# Autodesk Inventor assembly: Portalfraese_V2_Z-Axis
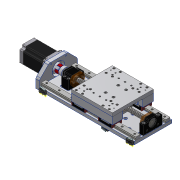
[picture p0: Inventor's stored thumbnail of the model, 180x180]
Saved by Autodesk Inventor 2016 (Build 200138000, 138)
## iProperties
Created: 2015-07-20
Part Number: Portalfraese_V2_Z-Axis
Document SubType Name: Assembly
Mass: 4544.64 g
Surface Area: 3288.98 cm^2
Volume: 1436.27 cm^3
Density: 3.16419 g/cm^3
## Documents named in this file (22)
- E:\GitHub\CNC-Router_Z-Axis\CNC-Router_Z-Axis.iam
- E:\GitHub\CNC-Router_Z-Axis\Linearfuehrung Bosch Rexroth R0442.iam
- E:\GitHub\CNC-Router_Z-Axis\ISSOKU_Ballscrew_D12x160_05_590104-13.iam
- E:\GitHub\CNC-Router_Z-Axis\Grundplatte.ipt
- E:\GitHub\Buy-Parts\Stepper_Nema23_23HS33-4008S.ipt
- E:\GitHub\CNC-Router_Z-Axis\Motorhalterung.ipt
- E:\GitHub\Buy-Parts\Klauenkupplung_d6-35_d8.ipt
- E:\GitHub\CNC-Router_Z-Axis\Schlitten.iam
- E:\GitHub\Standard-Parts\Zyl-Schr_ISO 4762 - M4 x 12_St-Vzkt.ipt
- E:\GitHub\Standard-Parts\Zyl-Schr_ISO 4762 - M3 x 35_INOX.ipt
- E:\GitHub\Standard-Parts\Zyl-Schr_ISO 4762 - M3 x 10_St-Vzkt.ipt
- E:\GitHub\Standard-Parts\U-Scheibe_ISO 7089 - 4 - 140 HV_St-Vzkt.ipt
- E:\GitHub\Standard-Parts\U-Scheibe_ISO 7089 - 6 - 140 HV_St-Vzkt.ipt
- E:\GitHub\Standard-Parts\Zyl-Schr_ISO 4762 - M6 x 20_St-Vzkt.ipt
- E:\GitHub\Standard-Parts\Zyl-Schr_ISO 4762 - M4 x 30_St-Vzkt.ipt
- E:\GitHub\Standard-Parts\Zyl-Schr_ISO 4762 - M5 x 30_St-Vzkt.ipt
- E:\GitHub\Buy-Parts\Microswitch Dongnan KW4A (S).ipt
- E:\GitHub\Buy-Parts\Klebesockel_HC-101SBK.ipt
- E:\GitHub\Buy-Parts\Micro_Mate-N-Lok_TE-Connectivity_3mm_1x4_Female.iam
- E:\GitHub\Buy-Parts\Micro_Mate-N-Lok_TE-Connectivity_3mm_2x2_Female.iam
- E:\GitHub\CNC-Router_Z-Axis\Zyl-Schr_ISO 4762 - M2 x 10_St-B.iam
- E:\GitHub\Standard-Parts\U-Scheibe_DIN 125 - A 2.2.ipt
## Components (86 placed, 21 different names)
1. ISSOKU_Ballscrew_D12x160_05_590104-13:1 [sub-assembly] — Mate:3, Mate:5, Mate:8, Insert:1, Mate:16, Mate:17, Flush:12, Mate:22, Insert:52, Insert:53, Insert:54, Insert:55, Insert:56, Insert:57
2. Linearfuehrung Bosch Rexroth R0442:1 [sub-assembly] — Mate:4, Flush:8, Mate:21, Mate:23, Mate:27, Insert:24, Insert:25, Insert:26, Insert:27, Insert:36, Insert:37, Insert:38, Insert:39
3. Linearfuehrung Bosch Rexroth R0442:2 [sub-assembly] — Mate:24, Mate:26, Mate:28, Mate:29, Mate:30, Insert:28, Insert:29, Insert:30, Insert:31, Insert:32, Insert:33, Insert:34, Insert:35
4. Grundplatte:1 — Mate:3, Mate:4, Flush:8, Mate:5, Angle:1, Mate:10, Flush:10, Mate:16, Mate:23, Mate:24, Mate:28, Insert:58, Insert:59, Mate:31, Mate:32, Mate:33, Insert:60, Mate:34, Mate:35, Insert:61, Mate:36, Flush:13, Mate:37, Mate:38, Mate:39, Mate:40
5. Stepper_Nema23_23HS33-4008S:1 — Mate:8, Angle:1, Mate:11, Mate:14, Insert:40, Insert:41, Insert:42, Insert:43
6. Motorhalterung:1 — Mate:10, Mate:11, Flush:10, Mate:14, Mate:26, Insert:50, Insert:51, Flush:16, Flush:17
7. Klauenkupplung_d6-35_d8:1 — Insert:1
8. Schlitten:1 [sub-assembly] — Mate:17, Flush:12, Mate:21, Mate:22, Mate:27, Mate:29, Mate:30, Insert:8, Insert:9, Insert:10, Insert:11, Insert:12, Insert:13, Insert:14, Insert:15, Insert:16, Insert:17, Insert:18, Insert:19, Insert:20, Insert:21, Insert:22, Insert:23
9. Zyl-Schr_ISO 4762 - M4 x 12_St-Vzkt:1
10. Zyl-Schr_ISO 4762 - M4 x 12_St-Vzkt:2
11. Zyl-Schr_ISO 4762 - M4 x 12_St-Vzkt:3
12. Zyl-Schr_ISO 4762 - M4 x 12_St-Vzkt:4
13. Zyl-Schr_ISO 4762 - M3 x 35_INOX:1 — Insert:8
14. Zyl-Schr_ISO 4762 - M3 x 35_INOX:2 — Insert:9
15. Zyl-Schr_ISO 4762 - M3 x 35_INOX:3 — Insert:11
16. Zyl-Schr_ISO 4762 - M3 x 35_INOX:4 — Insert:13
17. Zyl-Schr_ISO 4762 - M3 x 35_INOX:5 — Insert:12
18. Zyl-Schr_ISO 4762 - M3 x 35_INOX:6 — Insert:10
19. Zyl-Schr_ISO 4762 - M3 x 35_INOX:7 — Insert:15
20. Zyl-Schr_ISO 4762 - M3 x 35_INOX:8 — Insert:16
21. Zyl-Schr_ISO 4762 - M3 x 35_INOX:9 — Insert:14
22. Zyl-Schr_ISO 4762 - M3 x 35_INOX:10 — Insert:19
23. Zyl-Schr_ISO 4762 - M3 x 35_INOX:11 — Insert:23
24. Zyl-Schr_ISO 4762 - M3 x 35_INOX:12 — Insert:17
25. Zyl-Schr_ISO 4762 - M3 x 35_INOX:13 — Insert:21
26. Zyl-Schr_ISO 4762 - M3 x 35_INOX:14 — Insert:22
27. Zyl-Schr_ISO 4762 - M3 x 35_INOX:15 — Insert:18
28. Zyl-Schr_ISO 4762 - M3 x 35_INOX:16 — Insert:20
29. Zyl-Schr_ISO 4762 - M3 x 10_St-Vzkt:1 — Insert:28
30. Zyl-Schr_ISO 4762 - M3 x 10_St-Vzkt:2 — Insert:29
31. Zyl-Schr_ISO 4762 - M3 x 10_St-Vzkt:3 — Insert:30
32. Zyl-Schr_ISO 4762 - M3 x 10_St-Vzkt:4 — Insert:31
33. Zyl-Schr_ISO 4762 - M3 x 10_St-Vzkt:5 — Insert:32
34. Zyl-Schr_ISO 4762 - M3 x 10_St-Vzkt:6 — Insert:33
35. Zyl-Schr_ISO 4762 - M3 x 10_St-Vzkt:7 — Insert:34
36. Zyl-Schr_ISO 4762 - M3 x 10_St-Vzkt:8 — Insert:35
37. Zyl-Schr_ISO 4762 - M3 x 10_St-Vzkt:9 — Insert:24
38. Zyl-Schr_ISO 4762 - M3 x 10_St-Vzkt:10 — Insert:25
39. Zyl-Schr_ISO 4762 - M3 x 10_St-Vzkt:11 — Insert:26
40. Zyl-Schr_ISO 4762 - M3 x 10_St-Vzkt:12 — Insert:27
41. Zyl-Schr_ISO 4762 - M3 x 10_St-Vzkt:13 — Insert:36
42. Zyl-Schr_ISO 4762 - M3 x 10_St-Vzkt:14 — Insert:37
43. Zyl-Schr_ISO 4762 - M3 x 10_St-Vzkt:15 — Insert:38
44. Zyl-Schr_ISO 4762 - M3 x 10_St-Vzkt:16 — Insert:39
45. Zyl-Schr_ISO 4762 - M4 x 12_St-Vzkt:5 — Insert:44
46. U-Scheibe_ISO 7089 - 4 - 140 HV_St-Vzkt:1 — Insert:40, Insert:44
47. U-Scheibe_ISO 7089 - 4 - 140 HV_St-Vzkt:2 — Insert:41, Insert:45
48. U-Scheibe_ISO 7089 - 4 - 140 HV_St-Vzkt:3 — Insert:42, Insert:46
49. U-Scheibe_ISO 7089 - 4 - 140 HV_St-Vzkt:4 — Insert:43, Insert:47
50. Zyl-Schr_ISO 4762 - M4 x 12_St-Vzkt:6 — Insert:45
51. Zyl-Schr_ISO 4762 - M4 x 12_St-Vzkt:7 — Insert:46
52. Zyl-Schr_ISO 4762 - M4 x 12_St-Vzkt:8 — Insert:47
53. U-Scheibe_ISO 7089 - 6 - 140 HV_St-Vzkt:1 — Insert:48, Insert:50
54. Zyl-Schr_ISO 4762 - M6 x 20_St-Vzkt:1 — Insert:48
55. U-Scheibe_ISO 7089 - 6 - 140 HV_St-Vzkt:2 — Insert:51
56. Zyl-Schr_ISO 4762 - M6 x 20_St-Vzkt:2
57. Zyl-Schr_ISO 4762 - M4 x 30_St-Vzkt:1 — Insert:52
58. Zyl-Schr_ISO 4762 - M4 x 30_St-Vzkt:2 — Insert:53
59. Zyl-Schr_ISO 4762 - M4 x 30_St-Vzkt:3 — Insert:54
60. Zyl-Schr_ISO 4762 - M4 x 30_St-Vzkt:4 — Insert:55
61. Zyl-Schr_ISO 4762 - M5 x 30_St-Vzkt:1 — Insert:56
62. Zyl-Schr_ISO 4762 - M5 x 30_St-Vzkt:2 — Insert:57
63. Microswitch Dongnan KW4A (S):1 — Mate:35, Insert:61, Insert:68, Insert:69
64. Microswitch Dongnan KW4A (S):2 — Insert:60, Mate:34, Insert:66, Insert:67
65. Microswitch Dongnan KW4A (S):3 — Insert:58, Mate:32, Mate:33, Insert:74, Insert:75
66. Microswitch Dongnan KW4A (S):4 — Insert:59, Mate:31, Insert:76, Insert:77
67. Klebesockel_HC-101SBK:1 — Mate:36, Flush:13, Mate:37
68. Micro_Mate-N-Lok_TE-Connectivity_3mm_1x4_Female:1 [sub-assembly] — Mate:39, Mate:41, Mate:42, Flush:14, Flush:15
69. Micro_Mate-N-Lok_TE-Connectivity_3mm_2x2_Female:1 [sub-assembly] — Mate:40, Mate:42, Flush:14, Flush:16, Flush:17
70. Micro_Mate-N-Lok_TE-Connectivity_3mm_1x4_Female:2 [sub-assembly] — Mate:38, Mate:41, Flush:15
71. Zyl-Schr_ISO 4762 - M2 x 10_St-B:1 [sub-assembly] — Insert:62
72. U-Scheibe_DIN 125 - A 2.2:1 — Insert:62, Insert:67
73. Zyl-Schr_ISO 4762 - M2 x 10_St-B:2 [sub-assembly]
74. U-Scheibe_DIN 125 - A 2.2:2 — Insert:66
75. Zyl-Schr_ISO 4762 - M2 x 10_St-B:3 [sub-assembly]
76. U-Scheibe_DIN 125 - A 2.2:3 — Insert:68
77. Zyl-Schr_ISO 4762 - M2 x 10_St-B:4 [sub-assembly]
78. U-Scheibe_DIN 125 - A 2.2:4 — Insert:69
79. Zyl-Schr_ISO 4762 - M2 x 10_St-B:5 [sub-assembly]
80. U-Scheibe_DIN 125 - A 2.2:5 — Insert:74
81. Zyl-Schr_ISO 4762 - M2 x 10_St-B:6 [sub-assembly]
82. U-Scheibe_DIN 125 - A 2.2:6 — Insert:75
83. Zyl-Schr_ISO 4762 - M2 x 10_St-B:7 [sub-assembly]
84. U-Scheibe_DIN 125 - A 2.2:7 — Insert:76
85. Zyl-Schr_ISO 4762 - M2 x 10_St-B:8 [sub-assembly]
86. U-Scheibe_DIN 125 - A 2.2:8 — Insert:77
## Relationships (114: Insert 75, Mate 30, Flush 8, Angle 1)
- Mate:3: ISSOKU_Ballscrew_D12x160_05_590104-13:1 ↔ Grundplatte:1
- Mate:4: Linearfuehrung Bosch Rexroth R0442:1 ↔ Grundplatte:1
- Flush:8: Linearfuehrung Bosch Rexroth R0442:1 ↔ Grundplatte:1
- Mate:5 (3 mm): ISSOKU_Ballscrew_D12x160_05_590104-13:1 ↔ Grundplatte:1
- Mate:8: ISSOKU_Ballscrew_D12x160_05_590104-13:1 ↔ Stepper_Nema23_23HS33-4008S:1
- Angle:1 (0 deg): Grundplatte:1 ↔ Stepper_Nema23_23HS33-4008S:1
- Mate:10: Grundplatte:1 ↔ Motorhalterung:1
- Mate:11: Stepper_Nema23_23HS33-4008S:1 ↔ Motorhalterung:1
- Flush:10: Grundplatte:1 ↔ Motorhalterung:1
- Insert:1 (1.5 mm): ISSOKU_Ballscrew_D12x160_05_590104-13:1 ↔ Klauenkupplung_d6-35_d8:1
- Mate:14: Stepper_Nema23_23HS33-4008S:1 ↔ Motorhalterung:1
- Mate:16: ISSOKU_Ballscrew_D12x160_05_590104-13:1 ↔ Grundplatte:1
- Mate:17: ISSOKU_Ballscrew_D12x160_05_590104-13:1 ↔ Schlitten:1
- Flush:12: ISSOKU_Ballscrew_D12x160_05_590104-13:1 ↔ Schlitten:1
- Mate:21: Linearfuehrung Bosch Rexroth R0442:1 ↔ Schlitten:1
- Mate:22: ISSOKU_Ballscrew_D12x160_05_590104-13:1 ↔ Schlitten:1
- Mate:23: Linearfuehrung Bosch Rexroth R0442:1 ↔ Grundplatte:1
- Mate:24: Linearfuehrung Bosch Rexroth R0442:2 ↔ Grundplatte:1
- Mate:26: Linearfuehrung Bosch Rexroth R0442:2 ↔ Motorhalterung:1
- Mate:27: Linearfuehrung Bosch Rexroth R0442:1 ↔ Schlitten:1
- Mate:28: Linearfuehrung Bosch Rexroth R0442:2 ↔ Grundplatte:1
- Mate:29: Linearfuehrung Bosch Rexroth R0442:2 ↔ Schlitten:1
- Mate:30: Linearfuehrung Bosch Rexroth R0442:2 ↔ Schlitten:1
- [Insert]: Schlitten:1 ↔ Zyl-Schr_ISO 4762 - M4 x 12_St-Vzkt:1
- [Insert]: Schlitten:1 ↔ Zyl-Schr_ISO 4762 - M4 x 12_St-Vzkt:2
- [Insert]: Schlitten:1 ↔ Zyl-Schr_ISO 4762 - M4 x 12_St-Vzkt:4
- [Insert]: Schlitten:1 ↔ Zyl-Schr_ISO 4762 - M4 x 12_St-Vzkt:3
- Insert:8: Schlitten:1 ↔ Zyl-Schr_ISO 4762 - M3 x 35_INOX:1
- Insert:9: Schlitten:1 ↔ Zyl-Schr_ISO 4762 - M3 x 35_INOX:2
- Insert:10: Schlitten:1 ↔ Zyl-Schr_ISO 4762 - M3 x 35_INOX:6
- Insert:11: Schlitten:1 ↔ Zyl-Schr_ISO 4762 - M3 x 35_INOX:3
- Insert:12: Schlitten:1 ↔ Zyl-Schr_ISO 4762 - M3 x 35_INOX:5
- Insert:13: Schlitten:1 ↔ Zyl-Schr_ISO 4762 - M3 x 35_INOX:4
- Insert:14: Schlitten:1 ↔ Zyl-Schr_ISO 4762 - M3 x 35_INOX:9
- Insert:15: Schlitten:1 ↔ Zyl-Schr_ISO 4762 - M3 x 35_INOX:7
- Insert:16: Schlitten:1 ↔ Zyl-Schr_ISO 4762 - M3 x 35_INOX:8
- Insert:17: Schlitten:1 ↔ Zyl-Schr_ISO 4762 - M3 x 35_INOX:12
- Insert:18: Schlitten:1 ↔ Zyl-Schr_ISO 4762 - M3 x 35_INOX:15
- Insert:19: Schlitten:1 ↔ Zyl-Schr_ISO 4762 - M3 x 35_INOX:10
- Insert:20: Schlitten:1 ↔ Zyl-Schr_ISO 4762 - M3 x 35_INOX:16
- Insert:21: Schlitten:1 ↔ Zyl-Schr_ISO 4762 - M3 x 35_INOX:13
- Insert:22: Schlitten:1 ↔ Zyl-Schr_ISO 4762 - M3 x 35_INOX:14
- Insert:23: Schlitten:1 ↔ Zyl-Schr_ISO 4762 - M3 x 35_INOX:11
- Insert:24: Linearfuehrung Bosch Rexroth R0442:1 ↔ Zyl-Schr_ISO 4762 - M3 x 10_St-Vzkt:9
- Insert:25: Linearfuehrung Bosch Rexroth R0442:1 ↔ Zyl-Schr_ISO 4762 - M3 x 10_St-Vzkt:10
- Insert:26: Linearfuehrung Bosch Rexroth R0442:1 ↔ Zyl-Schr_ISO 4762 - M3 x 10_St-Vzkt:11
- Insert:27: Linearfuehrung Bosch Rexroth R0442:1 ↔ Zyl-Schr_ISO 4762 - M3 x 10_St-Vzkt:12
- Insert:28: Linearfuehrung Bosch Rexroth R0442:2 ↔ Zyl-Schr_ISO 4762 - M3 x 10_St-Vzkt:1
- Insert:29: Linearfuehrung Bosch Rexroth R0442:2 ↔ Zyl-Schr_ISO 4762 - M3 x 10_St-Vzkt:2
- Insert:30: Linearfuehrung Bosch Rexroth R0442:2 ↔ Zyl-Schr_ISO 4762 - M3 x 10_St-Vzkt:3
- Insert:31: Linearfuehrung Bosch Rexroth R0442:2 ↔ Zyl-Schr_ISO 4762 - M3 x 10_St-Vzkt:4
- Insert:32: Linearfuehrung Bosch Rexroth R0442:2 ↔ Zyl-Schr_ISO 4762 - M3 x 10_St-Vzkt:5
- Insert:33: Linearfuehrung Bosch Rexroth R0442:2 ↔ Zyl-Schr_ISO 4762 - M3 x 10_St-Vzkt:6
- Insert:34: Linearfuehrung Bosch Rexroth R0442:2 ↔ Zyl-Schr_ISO 4762 - M3 x 10_St-Vzkt:7
- Insert:35: Linearfuehrung Bosch Rexroth R0442:2 ↔ Zyl-Schr_ISO 4762 - M3 x 10_St-Vzkt:8
- Insert:36: Linearfuehrung Bosch Rexroth R0442:1 ↔ Zyl-Schr_ISO 4762 - M3 x 10_St-Vzkt:13
- Insert:37: Linearfuehrung Bosch Rexroth R0442:1 ↔ Zyl-Schr_ISO 4762 - M3 x 10_St-Vzkt:14
- Insert:38: Linearfuehrung Bosch Rexroth R0442:1 ↔ Zyl-Schr_ISO 4762 - M3 x 10_St-Vzkt:15
- Insert:39: Linearfuehrung Bosch Rexroth R0442:1 ↔ Zyl-Schr_ISO 4762 - M3 x 10_St-Vzkt:16
- Insert:40: Stepper_Nema23_23HS33-4008S:1 ↔ U-Scheibe_ISO 7089 - 4 - 140 HV_St-Vzkt:1
- Insert:41: Stepper_Nema23_23HS33-4008S:1 ↔ U-Scheibe_ISO 7089 - 4 - 140 HV_St-Vzkt:2
- Insert:42: Stepper_Nema23_23HS33-4008S:1 ↔ U-Scheibe_ISO 7089 - 4 - 140 HV_St-Vzkt:3
- Insert:43: Stepper_Nema23_23HS33-4008S:1 ↔ U-Scheibe_ISO 7089 - 4 - 140 HV_St-Vzkt:4
- Insert:44: Zyl-Schr_ISO 4762 - M4 x 12_St-Vzkt:5 ↔ U-Scheibe_ISO 7089 - 4 - 140 HV_St-Vzkt:1
- Insert:45: U-Scheibe_ISO 7089 - 4 - 140 HV_St-Vzkt:2 ↔ Zyl-Schr_ISO 4762 - M4 x 12_St-Vzkt:6
- Insert:46: U-Scheibe_ISO 7089 - 4 - 140 HV_St-Vzkt:3 ↔ Zyl-Schr_ISO 4762 - M4 x 12_St-Vzkt:7
- Insert:47: U-Scheibe_ISO 7089 - 4 - 140 HV_St-Vzkt:4 ↔ Zyl-Schr_ISO 4762 - M4 x 12_St-Vzkt:8
- Insert:48: U-Scheibe_ISO 7089 - 6 - 140 HV_St-Vzkt:1 ↔ Zyl-Schr_ISO 4762 - M6 x 20_St-Vzkt:1
- [Insert]: U-Scheibe_ISO 7089 - 6 - 140 HV_St-Vzkt:2 ↔ Zyl-Schr_ISO 4762 - M6 x 20_St-Vzkt:2
- Insert:50: Motorhalterung:1 ↔ U-Scheibe_ISO 7089 - 6 - 140 HV_St-Vzkt:1
- Insert:51: Motorhalterung:1 ↔ U-Scheibe_ISO 7089 - 6 - 140 HV_St-Vzkt:2
- Insert:52: ISSOKU_Ballscrew_D12x160_05_590104-13:1 ↔ Zyl-Schr_ISO 4762 - M4 x 30_St-Vzkt:1
- Insert:53: ISSOKU_Ballscrew_D12x160_05_590104-13:1 ↔ Zyl-Schr_ISO 4762 - M4 x 30_St-Vzkt:2
- Insert:54: ISSOKU_Ballscrew_D12x160_05_590104-13:1 ↔ Zyl-Schr_ISO 4762 - M4 x 30_St-Vzkt:3
- Insert:55: ISSOKU_Ballscrew_D12x160_05_590104-13:1 ↔ Zyl-Schr_ISO 4762 - M4 x 30_St-Vzkt:4
- Insert:56: ISSOKU_Ballscrew_D12x160_05_590104-13:1 ↔ Zyl-Schr_ISO 4762 - M5 x 30_St-Vzkt:1
- Insert:57: ISSOKU_Ballscrew_D12x160_05_590104-13:1 ↔ Zyl-Schr_ISO 4762 - M5 x 30_St-Vzkt:2
- Insert:58: Grundplatte:1 ↔ Microswitch Dongnan KW4A (S):3
- Insert:59: Grundplatte:1 ↔ Microswitch Dongnan KW4A (S):4
- Mate:31: Grundplatte:1 ↔ Microswitch Dongnan KW4A (S):4
- Mate:32: Grundplatte:1 ↔ Microswitch Dongnan KW4A (S):3
- Mate:33: Grundplatte:1 ↔ Microswitch Dongnan KW4A (S):3
- Insert:60: Grundplatte:1 ↔ Microswitch Dongnan KW4A (S):2
- Mate:34: Grundplatte:1 ↔ Microswitch Dongnan KW4A (S):2
- Mate:35: Grundplatte:1 ↔ Microswitch Dongnan KW4A (S):1
- Insert:61: Grundplatte:1 ↔ Microswitch Dongnan KW4A (S):1
- Mate:36: Grundplatte:1 ↔ Klebesockel_HC-101SBK:1
- Flush:13 (125 mm): Grundplatte:1 ↔ Klebesockel_HC-101SBK:1
- Mate:37: Grundplatte:1 ↔ Klebesockel_HC-101SBK:1
- Mate:38 (2 mm): Grundplatte:1 ↔ Micro_Mate-N-Lok_TE-Connectivity_3mm_1x4_Female:2
- Mate:39 (2 mm): Grundplatte:1 ↔ Micro_Mate-N-Lok_TE-Connectivity_3mm_1x4_Female:1
- Mate:40 (2 mm): Grundplatte:1 ↔ Micro_Mate-N-Lok_TE-Connectivity_3mm_2x2_Female:1
- Mate:41 (2 mm): Micro_Mate-N-Lok_TE-Connectivity_3mm_1x4_Female:1 ↔ Micro_Mate-N-Lok_TE-Connectivity_3mm_1x4_Female:2
- Mate:42 (2 mm): Micro_Mate-N-Lok_TE-Connectivity_3mm_1x4_Female:1 ↔ Micro_Mate-N-Lok_TE-Connectivity_3mm_2x2_Female:1
- Flush:14: Micro_Mate-N-Lok_TE-Connectivity_3mm_1x4_Female:1 ↔ Micro_Mate-N-Lok_TE-Connectivity_3mm_2x2_Female:1
- Flush:15: Micro_Mate-N-Lok_TE-Connectivity_3mm_1x4_Female:1 ↔ Micro_Mate-N-Lok_TE-Connectivity_3mm_1x4_Female:2
- Flush:16 (20 mm): Motorhalterung:1 ↔ Micro_Mate-N-Lok_TE-Connectivity_3mm_2x2_Female:1
- Flush:17 (50 mm): Motorhalterung:1 ↔ Micro_Mate-N-Lok_TE-Connectivity_3mm_2x2_Female:1
- Insert:62: Zyl-Schr_ISO 4762 - M2 x 10_St-B:1 ↔ U-Scheibe_DIN 125 - A 2.2:1
- [Insert]: Zyl-Schr_ISO 4762 - M2 x 10_St-B:2 ↔ U-Scheibe_DIN 125 - A 2.2:2
- [Insert]: Zyl-Schr_ISO 4762 - M2 x 10_St-B:3 ↔ U-Scheibe_DIN 125 - A 2.2:3
- [Insert]: Zyl-Schr_ISO 4762 - M2 x 10_St-B:4 ↔ U-Scheibe_DIN 125 - A 2.2:4
- Insert:66: Microswitch Dongnan KW4A (S):2 ↔ U-Scheibe_DIN 125 - A 2.2:2
- Insert:67: Microswitch Dongnan KW4A (S):2 ↔ U-Scheibe_DIN 125 - A 2.2:1
- Insert:68: Microswitch Dongnan KW4A (S):1 ↔ U-Scheibe_DIN 125 - A 2.2:3
- Insert:69: Microswitch Dongnan KW4A (S):1 ↔ U-Scheibe_DIN 125 - A 2.2:4
- [Insert]: Zyl-Schr_ISO 4762 - M2 x 10_St-B:5 ↔ U-Scheibe_DIN 125 - A 2.2:5
- [Insert]: Zyl-Schr_ISO 4762 - M2 x 10_St-B:6 ↔ U-Scheibe_DIN 125 - A 2.2:6
- [Insert]: Zyl-Schr_ISO 4762 - M2 x 10_St-B:7 ↔ U-Scheibe_DIN 125 - A 2.2:7
- [Insert]: Zyl-Schr_ISO 4762 - M2 x 10_St-B:8 ↔ U-Scheibe_DIN 125 - A 2.2:8
- Insert:74: Microswitch Dongnan KW4A (S):3 ↔ U-Scheibe_DIN 125 - A 2.2:5
- Insert:75: Microswitch Dongnan KW4A (S):3 ↔ U-Scheibe_DIN 125 - A 2.2:6
- Insert:76: Microswitch Dongnan KW4A (S):4 ↔ U-Scheibe_DIN 125 - A 2.2:7
- Insert:77: Microswitch Dongnan KW4A (S):4 ↔ U-Scheibe_DIN 125 - A 2.2:8
## Named parameters: d120_d119 = 0 mm, d161_d160 = 0 mm, d162_d160 = 0 mm, d163_d160 = 0 mm, d168_d160 = 0 mm, d169_d160 = 0 mm, d170_d160 = 0 mm, d171_d160 = 0 mm
